# Autodesk Inventor assembly: tr2
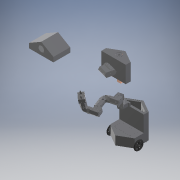
[picture p0: Inventor's stored thumbnail of the model, 180x180]
Saved by Autodesk Inventor 2017 (Build 210142000, 142)
## iProperties
Created: 2018-10-17
Part Number: tr2
Document SubType Name: Assembly
Designer: Administrator
Author: Administrator
## Documents named in this file (6)
- C:\Users\Dell\Documents\GitHub\tr2\TR2.iam
- C:\Users\Dell\Documents\GitHub\tr2\Base\Base.iam
- C:\Users\Dell\Documents\GitHub\tr2\Body\Body.iam
- C:\Users\Dell\Documents\GitHub\tr2\Arm\Arm.iam
- C:\Users\Dell\Documents\GitHub\tr2\Head\Head.iam
- C:\Users\Dell\Documents\GitHub\tr2\Body\CA01.ipt
## Components (5 placed, 5 different names)
1. Base:1 [sub-assembly] — Mate:2, Mate:9, Mate:27, Mate:28
2. Body:1 [sub-assembly] — Mate:9, Mate:22, Mate:23, Mate:24, Mate:25, Mate:26, Mate:27, Mate:28
3. Arm:1 [sub-assembly] — Mate:22, Mate:25, Mate:26
4. Head:1 [sub-assembly] — Mate:23, Mate:24
5. CA01:1
## Relationships (9: Mate 9)
- Mate:2 (50 mm): Base:1
- Mate:9: Base:1 ↔ Body:1
- Mate:22: Body:1 ↔ Arm:1
- Mate:23: Body:1 ↔ Head:1
- Mate:24: Body:1 ↔ Head:1
- Mate:25: Body:1 ↔ Arm:1
- Mate:26: Body:1 ↔ Arm:1
- Mate:27: Base:1 ↔ Body:1
- Mate:28: Base:1 ↔ Body:1
